# Autodesk Inventor assembly: Assembly1
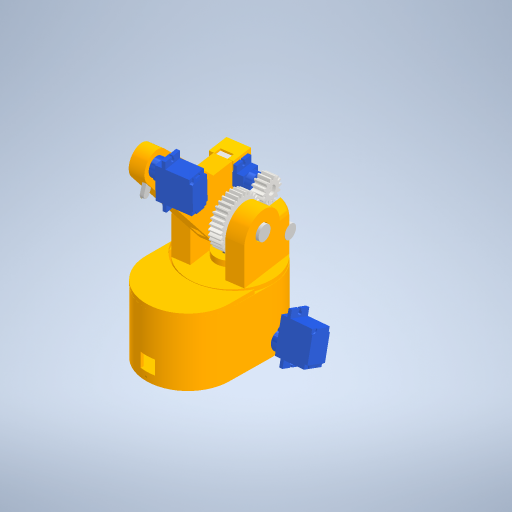
[picture p0: Inventor's stored thumbnail of the model, 512x512]
Saved by Autodesk Inventor 2024 (Build 280153000, 153)
## iProperties
Created: 2024-04-28
Part Number: Assembly1
Document SubType Name: Assembly
Designer: samue
Author: samue
## Documents named in this file (16)
- D:\samue\Escritorio\OneDrive - UVG\UVG\Año 2024\Semestre 1\Progra micros\Practicas\Brazo_robotico\Diseños 3D\Assembly1.iam
- D:\samue\Escritorio\OneDrive - UVG\UVG\Año 2024\Semestre 1\Progra micros\Practicas\Brazo_robotico\Diseños 3D\Servo SG90\Servo SG90.ipt
- D:\samue\Escritorio\OneDrive - UVG\UVG\Año 2024\Semestre 1\Progra micros\Practicas\Brazo_robotico\Diseños 3D\eje de motor.ipt
- D:\samue\Escritorio\OneDrive - UVG\UVG\Año 2024\Semestre 1\Progra micros\Practicas\Brazo_robotico\Diseños 3D\Brazo.ipt
- D:\samue\Escritorio\OneDrive - UVG\UVG\Año 2024\Semestre 1\Progra micros\Practicas\Brazo_robotico\Diseños 3D\EJE BRAZO.ipt
- D:\samue\Escritorio\OneDrive - UVG\UVG\Año 2024\Semestre 1\Progra micros\Practicas\Brazo_robotico\Diseños 3D\MG995\MG995.ipt
- D:\samue\Escritorio\OneDrive - UVG\UVG\Año 2024\Semestre 1\Progra micros\Practicas\Brazo_robotico\Diseños 3D\Base.ipt
- D:\samue\Escritorio\OneDrive - UVG\UVG\Año 2024\Semestre 1\Progra micros\Practicas\Brazo_robotico\Diseños 3D\base2.ipt
- D:\samue\Escritorio\OneDrive - UVG\UVG\Año 2024\Semestre 1\Progra micros\Practicas\Brazo_robotico\Diseños 3D\Assembly1\Design Accelerator\Spur Gears1.iam
- D:\samue\Escritorio\OneDrive - UVG\UVG\Año 2024\Semestre 1\Progra micros\Practicas\Brazo_robotico\Diseños 3D\Assembly1\Design Accelerator\Spur Gears2.iam
- D:\samue\Escritorio\OneDrive - UVG\UVG\Año 2024\Semestre 1\Progra micros\Practicas\Brazo_robotico\Diseños 3D\Tapa1.ipt
- D:\samue\Escritorio\OneDrive - UVG\UVG\Año 2024\Semestre 1\Progra micros\Practicas\Brazo_robotico\Diseños 3D\Assembly1\Design Accelerator\Spur Gears4.iam
- D:\samue\Escritorio\OneDrive - UVG\UVG\Año 2024\Semestre 1\Progra micros\Practicas\Brazo_robotico\Diseños 3D\EJE2.ipt
- D:\samue\Escritorio\OneDrive - UVG\UVG\Año 2024\Semestre 1\Progra micros\Practicas\Brazo_robotico\Diseños 3D\Sostiene motor.ipt
- D:\samue\Escritorio\OneDrive - UVG\UVG\Año 2024\Semestre 1\Progra micros\Practicas\Brazo_robotico\Diseños 3D\Tapa general.ipt
- D:\samue\Escritorio\OneDrive - UVG\UVG\Año 2024\Semestre 1\Progra micros\Practicas\Brazo_robotico\Diseños 3D\TAPA3.ipt
## Components (17 placed, 13 different names)
1. Servo SG90:1 — Rotational:1
2. eje de motor:1 — Rotational:1, Mate:1, Mate:2
3. Brazo:1 — Mate:1, Mate:2, Cylindrical:1, Rigid:2
4. EJE BRAZO:1 — Cylindrical:1, Mate:5, Mate:6
5. MG995:1 — Rigid:1
6. base2:1 — Mate:3, Mate:4, Rigid:1, Mate:5, Mate:8, Flush:4, Mate:9, Mate:15
7. Base:1 — Mate:3, Mate:4, Mate:12, Mate:13
8. Spur Gears:1 [sub-assembly] — Mate:6, Flush:1, Rigid:2, Flush:2
9. Spur Gears:2 [sub-assembly] — Flush:1, Flush:3, Rotational:2
10. Servo SG90:2 — Rotational:2, Mate:9, Mate:10, Mate:11
11. Tapa1:1
12. Servo SG90:3
13. Spur Gears:3 [sub-assembly] — Flush:2, Flush:3, Mate:7
14. EJE2:1 — Mate:7, Mate:8, Flush:4
15. Sostiene motor:1 — Mate:10, Mate:11, Mate:14
16. Tapa general:1 — Mate:12, Mate:13
17. TAPA3:1 — Mate:14, Mate:15
## Relationships (24: Mate 15, Flush 4, RevoluteJoint 2, WeldJoint 2, CylindricalJoint 1)
- Rotational:1 [RevoluteJoint] (1 mm): Servo SG90:1 ↔ eje de motor:1
- Mate:1: eje de motor:1 ↔ Brazo:1
- Mate:2: eje de motor:1 ↔ Brazo:1
- Cylindrical:1: Brazo:1 ↔ EJE BRAZO:1
- Mate:3: base2:1 ↔ Base:1
- Mate:4: base2:1 ↔ Base:1
- Rigid:1 [WeldJoint]: MG995:1 ↔ base2:1
- Mate:5: EJE BRAZO:1 ↔ base2:1
- Mate:6: EJE BRAZO:1 ↔ Spur Gears:1
- Flush:1: Spur Gears:1 ↔ Spur Gears:2
- Rigid:2 [WeldJoint]: Brazo:1 ↔ Spur Gears:1
- Flush:2: Spur Gears:1 ↔ Spur Gears:3
- Flush:3: Spur Gears:2 ↔ Spur Gears:3
- Mate:7: Spur Gears:3 ↔ EJE2:1
- Mate:8: base2:1 ↔ EJE2:1
- Flush:4: base2:1 ↔ EJE2:1
- Rotational:2 [RevoluteJoint]: Spur Gears:2 ↔ Servo SG90:2
- Mate:9: base2:1 ↔ Servo SG90:2
- Mate:10: Servo SG90:2 ↔ Sostiene motor:1
- Mate:11: Servo SG90:2 ↔ Sostiene motor:1
- Mate:12: Base:1 ↔ Tapa general:1
- Mate:13: Base:1 ↔ Tapa general:1
- Mate:14: Sostiene motor:1 ↔ TAPA3:1
- Mate:15: base2:1 ↔ TAPA3:1
